# Autodesk Inventor assembly: DriveBase Assembly
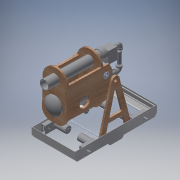
[picture p0: Inventor's stored thumbnail of the model, 180x180]
Saved by Autodesk Inventor 2018 (Build 220112000, 112)
## iProperties
Created: 2017-04-25
Part Number: DriveBase Assembly
Document SubType Name: Assembly
Designer: admin
Author: admin
## Documents named in this file (8)
- C:\Users\admin\Desktop\RoboEaglesCad2018\DriveBase Assembly.iam
- C:\Users\admin\Desktop\RoboEaglesCad2018\DriveBaseSidePanel.ipt
- C:\Users\admin\Desktop\RoboEaglesCad2018\DriveBaseFront.ipt
- C:\Users\admin\Desktop\RoboEaglesCad2018\Toughbox+Nano+All+Shafts+v2(ForUseInModel).iam
- C:\Users\admin\Desktop\RoboEaglesCad2018\InsideChurroBodySupport.ipt
- C:\Users\admin\Desktop\RoboEaglesCad2018\aFrameBase.ipt
- C:\Users\admin\Desktop\RoboEaglesCad2018\shooter.iam
- C:\Users\admin\Desktop\RoboEaglesCad2018\drivenAFrame.iam
## Components (13 placed, 7 different names)
1. DriveBaseSidePanel:1 — Flush:1, Flush:2, Mate:3, Mate:4, Mate:5, Mate:6, Flush:4, Flush:5, Mate:12, Mate:13, Insert:3, Insert:4, Angle:1, Angle:2
2. DriveBaseFront:1 — Flush:1, Flush:2, Mate:1, Mate:2, Mate:3, Mate:4, Mate:7, Mate:10
3. DriveBaseSidePanel:2 — Mate:1, Mate:2, Flush:3, Flush:6, Flush:7, Mate:11, Mate:14, Insert:1, Insert:2, Flush:8, Flush:9
4. DriveBaseFront:2 — Mate:5, Mate:6, Flush:3, Mate:8, Mate:9
5. Toughbox+Nano+All+Shafts+v2(ForUseInModel):1 [sub-assembly] — Flush:5, Mate:7, Mate:12
6. Toughbox+Nano+All+Shafts+v2(ForUseInModel):2 [sub-assembly] — Flush:4, Mate:8, Mate:13
7. Toughbox+Nano+All+Shafts+v2(ForUseInModel):3 [sub-assembly] — Flush:6, Mate:10, Mate:11
8. Toughbox+Nano+All+Shafts+v2(ForUseInModel):4 [sub-assembly] — Flush:7, Mate:9, Mate:14
9. InsideChurroBodySupport:1 — Insert:2, Insert:3, Angle:1
10. InsideChurroBodySupport:2 — Insert:1, Insert:4, Angle:2
11. aFrameBase:1 — Flush:8, Flush:9, Flush:10, Flush:11, Mate:15
12. shooter:1 [sub-assembly] — Mate:15
13. drivenAFrame:1 [sub-assembly] — Flush:10, Flush:11
## Relationships (32: Mate 15, Flush 11, Insert 4, Angle 2)
- Flush:1: DriveBaseSidePanel:1 ↔ DriveBaseFront:1
- Flush:2: DriveBaseSidePanel:1 ↔ DriveBaseFront:1
- Mate:1: DriveBaseFront:1 ↔ DriveBaseSidePanel:2
- Mate:2: DriveBaseFront:1 ↔ DriveBaseSidePanel:2
- Mate:3: DriveBaseSidePanel:1 ↔ DriveBaseFront:1
- Mate:4: DriveBaseSidePanel:1 ↔ DriveBaseFront:1
- Mate:5: DriveBaseSidePanel:1 ↔ DriveBaseFront:2
- Mate:6: DriveBaseSidePanel:1 ↔ DriveBaseFront:2
- Flush:3: DriveBaseSidePanel:2 ↔ DriveBaseFront:2
- Flush:4 (12.7 mm): DriveBaseSidePanel:1 ↔ Toughbox+Nano+All+Shafts+v2(ForUseInModel):2
- Flush:5 (12.7 mm): DriveBaseSidePanel:1 ↔ Toughbox+Nano+All+Shafts+v2(ForUseInModel):1
- Flush:6 (12.7 mm): DriveBaseSidePanel:2 ↔ Toughbox+Nano+All+Shafts+v2(ForUseInModel):3
- Flush:7 (12.7 mm): DriveBaseSidePanel:2 ↔ Toughbox+Nano+All+Shafts+v2(ForUseInModel):4
- Mate:7 (85.725 mm): DriveBaseFront:1 ↔ Toughbox+Nano+All+Shafts+v2(ForUseInModel):1
- Mate:8 (85.725 mm): DriveBaseFront:2 ↔ Toughbox+Nano+All+Shafts+v2(ForUseInModel):2
- Mate:9 (85.725 mm): DriveBaseFront:2 ↔ Toughbox+Nano+All+Shafts+v2(ForUseInModel):4
- Mate:10 (85.725 mm): DriveBaseFront:1 ↔ Toughbox+Nano+All+Shafts+v2(ForUseInModel):3
- Mate:11: DriveBaseSidePanel:2 ↔ Toughbox+Nano+All+Shafts+v2(ForUseInModel):3
- Mate:12: DriveBaseSidePanel:1 ↔ Toughbox+Nano+All+Shafts+v2(ForUseInModel):1
- Mate:13: DriveBaseSidePanel:1 ↔ Toughbox+Nano+All+Shafts+v2(ForUseInModel):2
- Mate:14: DriveBaseSidePanel:2 ↔ Toughbox+Nano+All+Shafts+v2(ForUseInModel):4
- Insert:1: DriveBaseSidePanel:2 ↔ InsideChurroBodySupport:2
- Insert:2: DriveBaseSidePanel:2 ↔ InsideChurroBodySupport:1
- Insert:3: DriveBaseSidePanel:1 ↔ InsideChurroBodySupport:1
- Insert:4: DriveBaseSidePanel:1 ↔ InsideChurroBodySupport:2
- Angle:1 (0 deg): DriveBaseSidePanel:1 ↔ InsideChurroBodySupport:1
- Angle:2 (0 deg): DriveBaseSidePanel:1 ↔ InsideChurroBodySupport:2
- Flush:8: DriveBaseSidePanel:2 ↔ aFrameBase:1
- Flush:9: DriveBaseSidePanel:2 ↔ aFrameBase:1
- Flush:10: aFrameBase:1 ↔ drivenAFrame:1
- Flush:11: aFrameBase:1 ↔ drivenAFrame:1
- Mate:15: aFrameBase:1 ↔ shooter:1
